# Autodesk Inventor assembly: CorteLaser
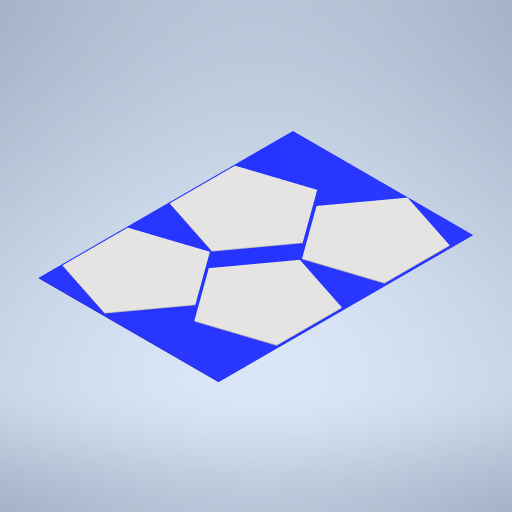
[picture p0: Inventor's stored thumbnail of the model, 512x512]
Saved by Autodesk Inventor 2024 (Build 280153000, 153)
## iProperties
Created: 2024-05-07
Part Number: CorteLaser
Document SubType Name: Assembly
Designer: sergi
Author: sergi
## Documents named in this file (3)
- C:\Users\sergi\OneDrive\Escritorio\proyectos\Piso\Dodecaedro\CorteLaser.iam
- C:\Users\sergi\OneDrive\Escritorio\proyectos\Piso\Dodecaedro\Plancha.ipt
- C:\Users\sergi\OneDrive\Escritorio\Pentagono\Pentagono.ipt
## Components (5 placed, 2 different names)
1. Plancha:1 — Coincidencia:1, Nivelación:1, Coincidencia:2, Nivelación:2, Coincidencia:3, Nivelación:3, Coincidencia:4, Nivelación:4
2. Pentagono:1 — Coincidencia:1, Nivelación:1
3. Pentagono:2 — Coincidencia:3, Nivelación:3
4. Pentagono:3 — Coincidencia:2, Nivelación:2
5. Pentagono:4 — Coincidencia:4, Nivelación:4
## Relationships (8: Mate 4, Flush 4)
- Coincidencia:1 [Mate]: Plancha:1 ↔ Pentagono:1
- Nivelación:1 [Flush] (3 mm): Plancha:1 ↔ Pentagono:1
- Coincidencia:2 [Mate]: Plancha:1 ↔ Pentagono:3
- Nivelación:2 [Flush] (3 mm): Plancha:1 ↔ Pentagono:3
- Coincidencia:3 [Mate]: Plancha:1 ↔ Pentagono:2
- Nivelación:3 [Flush] (3 mm): Plancha:1 ↔ Pentagono:2
- Coincidencia:4 [Mate]: Plancha:1 ↔ Pentagono:4
- Nivelación:4 [Flush] (3 mm): Plancha:1 ↔ Pentagono:4
